# Autodesk Inventor assembly: Leg Pair Assembly Spider Crab
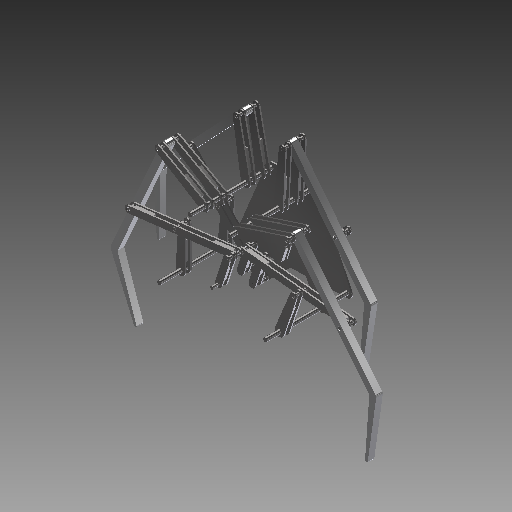
[picture p0: Inventor's stored thumbnail of the model, 512x512]
Saved by Autodesk Inventor 2019 (Build 230136000, 136)
## iProperties
Created: 2019-08-25
Part Number: Leg Pair Assembly Spider Crab
Document SubType Name: Assembly
Designer: DIBYOJYOTI
Mass: 1727.29 g
Surface Area: 1932.86 cm^2
Volume: 287.425 cm^3
Density: 6.00951 g/cm^3
Author: DIBYOJYOTI
## Documents named in this file (12)
- D:\TITO\Autocad\Leg Pair Assembly Spider Crab.iam
- D:\TITO\Autocad\Crank.ipt
- D:\TITO\Autocad\Leg Spider Crab.ipt
- D:\TITO\Autocad\Lower Rocker Arm Spider Crab.ipt
- D:\TITO\Autocad\Rocker arm Leg Spider Crab.ipt
- D:\TITO\Autocad\Upper Rocker Arm Spider Crab.ipt
- D:\TITO\Autocad\Joint Pin Spider Crab.ipt
- D:\TITO\Autocad\Short Joint Pin Spider Crab.ipt
- D:\TITO\Autocad\Long Joint Pin Spider Crab.ipt
- D:\TITO\Autocad\Upper Rod Spider Crab.ipt
- D:\TITO\Autocad\Crank Joint Pin Spider Crab.ipt
- D:\TITO\Autocad\Frame.ipt
## Components (51 placed, 11 different names)
1. Leg Spider Crab:1 — Insert:7, Insert:15
2. Rocker arm Leg Spider Crab:1 — Insert:13, Insert:14, Insert:17
3. Crank:1 — Insert:16, Insert:37, Flush:1
4. Joint Pin Spider Crab:1 — Insert:7, Insert:45, Insert:53
5. Short Joint Pin Spider Crab:2 — Insert:13, Insert:43
6. Short Joint Pin Spider Crab:3 — Insert:14, Insert:15
7. Long Joint Pin Spider Crab:1 — Insert:16, Insert:17, Insert:25, Insert:26
8. Leg Spider Crab:2
9. Rocker arm Leg Spider Crab:2 — Insert:25
10. Joint Pin Spider Crab:2 — Insert:49, Insert:51
11. Short Joint Pin Spider Crab:4 — Insert:47
12. Short Joint Pin Spider Crab:5
13. Crank:2 — Insert:26, Insert:36, Flush:1
14. Upper Rod Spider Crab:1 — Insert:42, Insert:46, Insert:54, Rigid:3
15. Upper Rod Spider Crab:2 — Insert:41, Insert:50, Insert:52, Rigid:4
16. Upper Rod Spider Crab:3 — Insert:39, Insert:44, Rigid:1
17. Upper Rod Spider Crab:4 — Insert:40, Insert:48, Rigid:2
18. Crank Joint Pin Spider Crab:1 — Insert:37, Rigid:5
19. Crank Joint Pin Spider Crab:2 — Insert:36, Insert:38, Rotational:1
20. Frame:1 — Insert:38, Insert:39, Insert:40, Insert:41, Insert:42, Rotational:1
21. Upper Rocker Arm Spider Crab:1 — Insert:53, Insert:54
22. Lower Rocker Arm Spider Crab:2 — Insert:43, Insert:44
23. Upper Rocker Arm Spider Crab:2 — Insert:45, Insert:46
24. Lower Rocker Arm Spider Crab:3 — Insert:47, Insert:48
25. Upper Rocker Arm Spider Crab:3 — Insert:49, Insert:50
26. Upper Rocker Arm Spider Crab:4 — Insert:51, Insert:52
27. Leg Spider Crab:3
28. Rocker arm Leg Spider Crab:3
29. Crank:3 — Insert:59
30. Joint Pin Spider Crab:3
31. Short Joint Pin Spider Crab:6
32. Short Joint Pin Spider Crab:7
33. Long Joint Pin Spider Crab:2 — Insert:59
34. Leg Spider Crab:4
35. Rocker arm Leg Spider Crab:4
36. Joint Pin Spider Crab:4
37. Short Joint Pin Spider Crab:8
38. Short Joint Pin Spider Crab:9
39. Crank:4
40. Upper Rod Spider Crab:5 — Rigid:3
41. Upper Rod Spider Crab:6 — Rigid:4
42. Upper Rod Spider Crab:7 — Rigid:1
43. Upper Rod Spider Crab:8 — Rigid:2
44. Crank Joint Pin Spider Crab:3
45. Crank Joint Pin Spider Crab:4 — Rigid:5
46. Upper Rocker Arm Spider Crab:5
47. Lower Rocker Arm Spider Crab:4
48. Upper Rocker Arm Spider Crab:6
49. Lower Rocker Arm Spider Crab:5
50. Upper Rocker Arm Spider Crab:7
51. Upper Rocker Arm Spider Crab:8
## Relationships (65: Insert 57, WeldJoint 5, Flush 2, RevoluteJoint 1)
- Insert:7 (-11 mm): Leg Spider Crab:1 ↔ Joint Pin Spider Crab:1
- Insert:13: Rocker arm Leg Spider Crab:1 ↔ Short Joint Pin Spider Crab:2
- Insert:14: Rocker arm Leg Spider Crab:1 ↔ Short Joint Pin Spider Crab:3
- Insert:15: Leg Spider Crab:1 ↔ Short Joint Pin Spider Crab:3
- Insert:16: Crank:1 ↔ Long Joint Pin Spider Crab:1
- Insert:17 (-22 mm): Rocker arm Leg Spider Crab:1 ↔ Long Joint Pin Spider Crab:1
- [Insert] (-11 mm): Leg Spider Crab:2 ↔ Joint Pin Spider Crab:2
- [Insert]: Rocker arm Leg Spider Crab:2 ↔ Short Joint Pin Spider Crab:4
- [Insert]: Rocker arm Leg Spider Crab:2 ↔ Short Joint Pin Spider Crab:5
- [Insert]: Leg Spider Crab:2 ↔ Short Joint Pin Spider Crab:5
- Insert:25 (11 mm): Long Joint Pin Spider Crab:1 ↔ Rocker arm Leg Spider Crab:2
- Insert:26: Long Joint Pin Spider Crab:1 ↔ Crank:2
- Insert:36: Crank:2 ↔ Crank Joint Pin Spider Crab:2
- Insert:37 (-10 mm): Crank:1 ↔ Crank Joint Pin Spider Crab:1
- Flush:1: Crank:1 ↔ Crank:2
- Insert:38 (-1 mm): Crank Joint Pin Spider Crab:2 ↔ Frame:1
- Insert:39 (-1 mm): Upper Rod Spider Crab:3 ↔ Frame:1
- Insert:40 (-1 mm): Upper Rod Spider Crab:4 ↔ Frame:1
- Insert:41 (-1 mm): Upper Rod Spider Crab:2 ↔ Frame:1
- Insert:42 (-1 mm): Upper Rod Spider Crab:1 ↔ Frame:1
- Rotational:1 [RevoluteJoint] (-1 mm): Crank Joint Pin Spider Crab:2 ↔ Frame:1
- Insert:43: Short Joint Pin Spider Crab:2 ↔ Lower Rocker Arm Spider Crab:2
- Insert:44 (21 mm): Upper Rod Spider Crab:3 ↔ Lower Rocker Arm Spider Crab:2
- Insert:45: Joint Pin Spider Crab:1 ↔ Upper Rocker Arm Spider Crab:2
- Insert:46 (10 mm): Upper Rod Spider Crab:1 ↔ Upper Rocker Arm Spider Crab:2
- Insert:47: Short Joint Pin Spider Crab:4 ↔ Lower Rocker Arm Spider Crab:3
- Insert:48 (21 mm): Upper Rod Spider Crab:4 ↔ Lower Rocker Arm Spider Crab:3
- Insert:49: Joint Pin Spider Crab:2 ↔ Upper Rocker Arm Spider Crab:3
- Insert:50 (10 mm): Upper Rod Spider Crab:2 ↔ Upper Rocker Arm Spider Crab:3
- Insert:51: Joint Pin Spider Crab:2 ↔ Upper Rocker Arm Spider Crab:4
- Insert:52 (21 mm): Upper Rod Spider Crab:2 ↔ Upper Rocker Arm Spider Crab:4
- Insert:53: Joint Pin Spider Crab:1 ↔ Upper Rocker Arm Spider Crab:1
- Insert:54 (21 mm): Upper Rod Spider Crab:1 ↔ Upper Rocker Arm Spider Crab:1
- [Insert] (-11 mm): Leg Spider Crab:3 ↔ Joint Pin Spider Crab:3
- [Insert]: Rocker arm Leg Spider Crab:3 ↔ Short Joint Pin Spider Crab:6
- [Insert]: Rocker arm Leg Spider Crab:3 ↔ Short Joint Pin Spider Crab:7
- [Insert]: Leg Spider Crab:3 ↔ Short Joint Pin Spider Crab:7
- Insert:59: Crank:3 ↔ Long Joint Pin Spider Crab:2
- [Insert] (-22 mm): Rocker arm Leg Spider Crab:3 ↔ Long Joint Pin Spider Crab:2
- [Insert] (-11 mm): Leg Spider Crab:4 ↔ Joint Pin Spider Crab:4
- [Insert]: Rocker arm Leg Spider Crab:4 ↔ Short Joint Pin Spider Crab:8
- [Insert]: Rocker arm Leg Spider Crab:4 ↔ Short Joint Pin Spider Crab:9
- [Insert]: Leg Spider Crab:4 ↔ Short Joint Pin Spider Crab:9
- [Insert] (11 mm): Long Joint Pin Spider Crab:2 ↔ Rocker arm Leg Spider Crab:4
- [Insert]: Long Joint Pin Spider Crab:2 ↔ Crank:4
- [Insert]: Crank:4 ↔ Crank Joint Pin Spider Crab:4
- [Insert] (-10 mm): Crank:3 ↔ Crank Joint Pin Spider Crab:3
- [Flush]: Crank:3 ↔ Crank:4
- [Insert]: Short Joint Pin Spider Crab:6 ↔ Lower Rocker Arm Spider Crab:4
- [Insert] (21 mm): Upper Rod Spider Crab:7 ↔ Lower Rocker Arm Spider Crab:4
- [Insert]: Joint Pin Spider Crab:3 ↔ Upper Rocker Arm Spider Crab:6
- [Insert] (10 mm): Upper Rod Spider Crab:5 ↔ Upper Rocker Arm Spider Crab:6
- [Insert]: Short Joint Pin Spider Crab:8 ↔ Lower Rocker Arm Spider Crab:5
- [Insert] (21 mm): Upper Rod Spider Crab:8 ↔ Lower Rocker Arm Spider Crab:5
- [Insert]: Joint Pin Spider Crab:4 ↔ Upper Rocker Arm Spider Crab:7
- [Insert] (10 mm): Upper Rod Spider Crab:6 ↔ Upper Rocker Arm Spider Crab:7
- [Insert]: Joint Pin Spider Crab:4 ↔ Upper Rocker Arm Spider Crab:8
- [Insert] (21 mm): Upper Rod Spider Crab:6 ↔ Upper Rocker Arm Spider Crab:8
- [Insert]: Joint Pin Spider Crab:3 ↔ Upper Rocker Arm Spider Crab:5
- [Insert] (21 mm): Upper Rod Spider Crab:5 ↔ Upper Rocker Arm Spider Crab:5
- Rigid:1 [WeldJoint]: Upper Rod Spider Crab:3 ↔ Upper Rod Spider Crab:7
- Rigid:2 [WeldJoint]: Upper Rod Spider Crab:4 ↔ Upper Rod Spider Crab:8
- Rigid:3 [WeldJoint]: Upper Rod Spider Crab:1 ↔ Upper Rod Spider Crab:5
- Rigid:4 [WeldJoint]: Upper Rod Spider Crab:2 ↔ Upper Rod Spider Crab:6
- Rigid:5 [WeldJoint]: Crank Joint Pin Spider Crab:1 ↔ Crank Joint Pin Spider Crab:4
## Named parameters: d36_d32 = 0 mm, d37_d33 = 0 mm, d39_d28 = 0 mm, d40_d16 = -11 mm, d114_d109 = 10 mm, d115_d110 = 0 mm, d116_d111 = 21 mm, d117_d112 = 0 mm, d118_d113 = 21 mm, d119_d103 = 21 mm, d120_d104 = 0 mm, d121_d105 = 10 mm, d122_d106 = 0 mm, d123_d107 = 21 mm, d124_d108 = 0 mm, d125_d102 = 0 mm, d126_d43 = 11 mm, d127_d44 = 0 mm, d128_d58 = 0 mm, d129_d59 = -10 mm, d130_d60 = 0 mm, d131_d16 = -11 mm, d132_d28 = 0 mm, d133_d32 = 0 mm, d134_d33 = 0 mm, d135_d34 = 0 mm, d136_d35 = -22 mm, d137_d36_d32 = 0 mm, d138_d37_d33 = 0 mm, d139_d39_d28 = 0 mm, d140_d40_d16 = -11 mm
